# Autodesk Inventor assembly: FullAssem
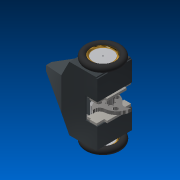
[picture p0: Inventor's stored thumbnail of the model, 180x180]
Saved by Autodesk Inventor 2019 (Build 230136000, 136)
## iProperties
Created: 2018-08-17
Part Number: FullAssem
Document SubType Name: Assembly
Designer: Kitte_X
Author: Kitte_X
## Documents named in this file (13)
- C:\Users\Kitte_X\Documents\Inventor\BattleBot\FullAssem.iam
- C:\Users\Kitte_X\Documents\Inventor\BattleBot\Guessed Dimensions\FrameThickBracket.ipt
- C:\Users\Kitte_X\Documents\Inventor\BattleBot\Guessed Dimensions\FrameThinBracket.ipt
- C:\Users\Kitte_X\Documents\Inventor\BattleBot\Guessed Dimensions\SpinnerAxelV1.ipt
- C:\Users\Kitte_X\Documents\Inventor\BattleBot\Guessed Dimensions\SpinnerV1.ipt
- C:\Users\Kitte_X\Documents\Inventor\BattleBot\battlebotspinner20mmplate.ipt
- C:\Users\Kitte_X\Documents\Inventor\BattleBot\battlebotupperframe.ipt
- C:\Users\Kitte_X\Documents\Inventor\BattleBot\Guessed Dimensions\FrameMainMotorMount.ipt
- C:\Users\Kitte_X\Documents\Inventor\BattleBot\Guessed Dimensions\drivemotors.ipt
- C:\Users\Kitte_X\Documents\Inventor\BattleBot\Guessed Dimensions\wheel.ipt
- C:\Users\Kitte_X\Documents\Inventor\BattleBot\armorMk1.ipt
- C:\Users\Kitte_X\Pictures\Screenshots\4249328706742569115.jpg
- C:\Users\Kitte_X\Pictures\Screenshots\X59KrzT.jpg
## Components (16 placed, 10 different names)
1. FrameThickBracket:1 — Mate:10, Mate:33, Mate:34, Mate:36, Flush:8
2. FrameThinBracket:1 — Mate:4, Mate:29, Mate:30, Flush:9
3. SpinnerAxelV1:1 — Mate:16, Mate:17, Mate:18, Mate:24, Mate:25
4. SpinnerV1:1 — Mate:24, Mate:25, Mate:26
5. battlebotspinner20mmplate:1 — Mate:13, Flush:3, Flush:4, Mate:16
6. battlebotupperframe:1 — Mate:1, Mate:4, Mate:7, Mate:10, Mate:13, Mate:14, Flush:1, Flush:2, Flush:3, Flush:4, Mate:22, Flush:7, Symmetry:1, Mate:44, Mate:45
7. battlebotspinner20mmplate:2 — Mate:14, Flush:1, Flush:2, Mate:15, Flush:5, Flush:6, Mate:17, Mate:18, Mate:26
8. battlebotupperframe:2 — Mate:15, Flush:5, Flush:6, Mate:23, Mate:27, Mate:28, Mate:29, Mate:30, Mate:31, Mate:32, Mate:33, Mate:34, Symmetry:1, Mate:43
9. FrameThickBracket:2 — Mate:1, Mate:27, Mate:28, Mate:35
10. FrameThinBracket:2 — Mate:7, Mate:31, Mate:32
11. FrameMainMotorMount:1 — Mate:22, Mate:23, Flush:7
12. drivemotors:1 — Mate:36, Flush:8, Mate:37, Mate:39, Mate:42
13. drivemotors:2 — Mate:35, Flush:9, Mate:37, Mate:38, Mate:40, Mate:41
14. wheel:1 — Mate:39, Mate:42
15. wheel:2 — Mate:40, Mate:41
16. armorMk1:1 — Mate:43, Mate:44, Mate:45
## Relationships (44: Mate 34, Flush 9, Symmetry 1)
- Mate:1: battlebotupperframe:1 ↔ FrameThickBracket:2
- Mate:4: FrameThinBracket:1 ↔ battlebotupperframe:1
- Mate:7: battlebotupperframe:1 ↔ FrameThinBracket:2
- Mate:10: FrameThickBracket:1 ↔ battlebotupperframe:1
- Mate:13: battlebotspinner20mmplate:1 ↔ battlebotupperframe:1
- Mate:14: battlebotupperframe:1 ↔ battlebotspinner20mmplate:2
- Flush:1: battlebotupperframe:1 ↔ battlebotspinner20mmplate:2
- Flush:2: battlebotupperframe:1 ↔ battlebotspinner20mmplate:2
- Flush:3: battlebotspinner20mmplate:1 ↔ battlebotupperframe:1
- Flush:4: battlebotspinner20mmplate:1 ↔ battlebotupperframe:1
- Mate:15: battlebotspinner20mmplate:2 ↔ battlebotupperframe:2
- Flush:5: battlebotspinner20mmplate:2 ↔ battlebotupperframe:2
- Flush:6: battlebotspinner20mmplate:2 ↔ battlebotupperframe:2
- Mate:16: SpinnerAxelV1:1 ↔ battlebotspinner20mmplate:1
- Mate:17: SpinnerAxelV1:1 ↔ battlebotspinner20mmplate:2
- Mate:18: SpinnerAxelV1:1 ↔ battlebotspinner20mmplate:2
- Mate:22: battlebotupperframe:1 ↔ FrameMainMotorMount:1
- Mate:23: battlebotupperframe:2 ↔ FrameMainMotorMount:1
- Flush:7 (123 mm): battlebotupperframe:1 ↔ FrameMainMotorMount:1
- Mate:24: SpinnerAxelV1:1 ↔ SpinnerV1:1
- Mate:25: SpinnerAxelV1:1 ↔ SpinnerV1:1
- Mate:26 (40 mm): SpinnerV1:1 ↔ battlebotspinner20mmplate:2
- Mate:27: battlebotupperframe:2 ↔ FrameThickBracket:2
- Mate:28: battlebotupperframe:2 ↔ FrameThickBracket:2
- Mate:29: FrameThinBracket:1 ↔ battlebotupperframe:2
- Mate:30: FrameThinBracket:1 ↔ battlebotupperframe:2
- Mate:31: battlebotupperframe:2 ↔ FrameThinBracket:2
- Mate:32: battlebotupperframe:2 ↔ FrameThinBracket:2
- Mate:33: FrameThickBracket:1 ↔ battlebotupperframe:2
- Mate:34: FrameThickBracket:1 ↔ battlebotupperframe:2
- Mate:35: FrameThickBracket:2 ↔ drivemotors:2
- Mate:36: FrameThickBracket:1 ↔ drivemotors:1
- Flush:8: FrameThickBracket:1 ↔ drivemotors:1
- Flush:9: FrameThinBracket:1 ↔ drivemotors:2
- Mate:37: drivemotors:1 ↔ drivemotors:2
- Symmetry:1: battlebotupperframe:1 ↔ battlebotupperframe:2
- Mate:38: drivemotors:2
- Mate:39: drivemotors:1 ↔ wheel:1
- Mate:40: drivemotors:2 ↔ wheel:2
- Mate:41: drivemotors:2 ↔ wheel:2
- Mate:42: drivemotors:1 ↔ wheel:1
- Mate:43: battlebotupperframe:2 ↔ armorMk1:1
- Mate:44: battlebotupperframe:1 ↔ armorMk1:1
- Mate:45: battlebotupperframe:1 ↔ armorMk1:1
